# Autodesk Inventor assembly: ChestController
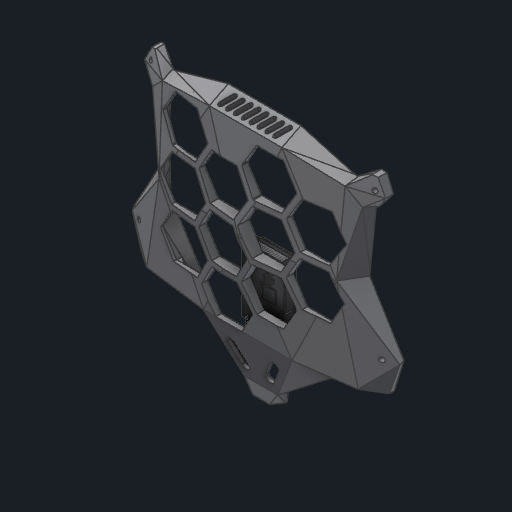
[picture p0: Inventor's stored thumbnail of the model, 512x512]
Saved by Autodesk Inventor 2023 (Build 270158000, 158)
## iProperties
Created: 2023-12-19
Part Number: ChestController
Document SubType Name: Assembly
Designer: valer
Author: valer
## Documents named in this file (3)
- C:\Users\valer\Desktop\str1ker\cad\ChestController.iam
- C:\Users\valer\Desktop\str1ker\cad\ControlBoard2.ipt
- C:\Users\valer\Desktop\str1ker\cad\external\ArduinoMegaRev3.ipt
## Components (2 placed, 2 different names)
1. ControlBoard2:1 — Flush:1, Flush:2
2. ArduinoMegaRev3:1 — Mate:1, Angle:1
## Relationships (4: Flush 2, Mate 1, Angle 1)
- Mate:1: ArduinoMegaRev3:1
- Angle:1 (180 deg): ArduinoMegaRev3:1
- Flush:1: ControlBoard2:1
- Flush:2: ControlBoard2:1
